# Autodesk Inventor assembly: TableAssembly
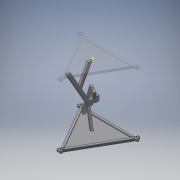
[picture p0: Inventor's stored thumbnail of the model, 180x180]
Saved by Autodesk Inventor 2018.3 (Build 223284000, 284)
## iProperties
Created: 2020-03-27
Part Number: TableAssembly
Document SubType Name: Assembly
Designer: Ivan
Author: Ivan
## Documents named in this file (3)
- C:\Users\Ivan\Documents\GitHub\Tensegrity-Imposible-Table\3D model\TableAssembly.iam
- C:\Users\Ivan\Documents\GitHub\Tensegrity-Imposible-Table\3D model\TableBaseWithHoles.ipt
- C:\Users\Ivan\Documents\GitHub\Tensegrity-Imposible-Table\3D model\TableSupport.ipt
## Components (4 placed, 2 different names)
1. TableBaseWithHoles:1 — Mate:1, Mate:2, Angle:1, Mate:6, Flush:1, Mate:7, Mate:8, Mate:9
2. TableSupport:1 — Mate:1, Mate:2, Mate:7
3. TableBaseWithHoles:2 — Mate:3, Mate:4, Mate:5, Angle:1, Mate:6, Flush:1, Mate:8, Mate:9
4. TableSupport:2 — Mate:3, Mate:4, Mate:5
## Relationships (11: Mate 9, Angle 1, Flush 1)
- Mate:1: TableBaseWithHoles:1 ↔ TableSupport:1
- Mate:2: TableBaseWithHoles:1 ↔ TableSupport:1
- Mate:3: TableBaseWithHoles:2 ↔ TableSupport:2
- Mate:4: TableBaseWithHoles:2 ↔ TableSupport:2
- Mate:5 (0.5 mm): TableBaseWithHoles:2 ↔ TableSupport:2
- Angle:1 (180 deg): TableBaseWithHoles:1 ↔ TableBaseWithHoles:2
- Mate:6 (155 mm): TableBaseWithHoles:1 ↔ TableBaseWithHoles:2
- Flush:1: TableBaseWithHoles:1 ↔ TableBaseWithHoles:2
- Mate:7 (0.5 mm): TableBaseWithHoles:1 ↔ TableSupport:1
- Mate:8: TableBaseWithHoles:1 ↔ TableBaseWithHoles:2
- Mate:9: TableBaseWithHoles:1 ↔ TableBaseWithHoles:2
